# Autodesk Inventor assembly: Direccion
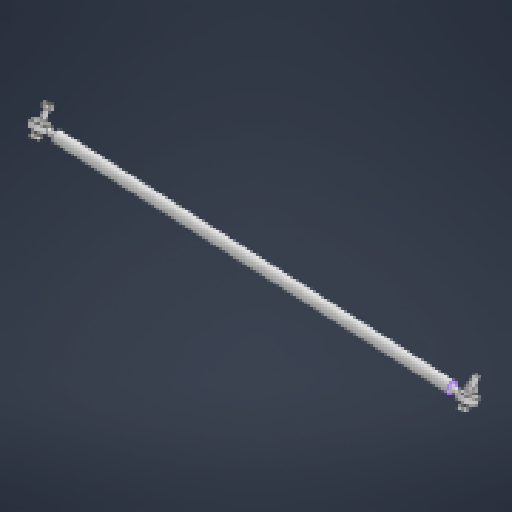
[picture p0: Inventor's stored thumbnail of the model, 512x512]
Saved by Autodesk Inventor 2024 (Build 280153000, 153)
## iProperties
Created: 2023-01-20
Part Number: Direccion
Document SubType Name: Assembly
Designer: juanj
Sending System: Autodesk Inventor 2023
Preprocessor: ST-DEVELOPER v19
Title: C:\Users\juanj\OneDrive\Documentos\Unisabana\Shell\C23 DESING\Dirección\Direccion.stp
Author: juanj
## Documents named in this file (5)
- C:\Users\juanj\Documents\Documentos\Unisabana\Shell\A23[F]\PFA23[F]\D23[F].iam
- C:\Users\juanj\Documents\Documentos\Unisabana\Shell\A23[F]\PWC\BarraAckerman.ipt
- C:\Users\juanj\Documents\Documentos\Unisabana\Shell\A23[F]\PWC\Rotula.ipt
- C:\Users\juanj\Documents\Documentos\Unisabana\Shell\A23[F]\PWC\Tornillo.ipt
- C:\Users\juanj\Documents\Documentos\Unisabana\Shell\A23[F]\PWC\Tuerca.ipt
## Components (7 placed, 4 different names)
1. BarraAckerman:1 — Insert:1, Insert:4
2. Rotula:1 — Insert:1, Insert:2, Insert:3
3. Tornillo:1 — Insert:5, Angle:1
4. Tornillo:2 — Insert:2, Angle:1
5. Tuerca:1 — Insert:6
6. Tuerca:2 — Insert:3
7. Rotula:2 — Insert:4, Insert:5, Insert:6
## Relationships (7: Insert 6, Angle 1)
- Insert:1 (-15 mm): BarraAckerman:1 ↔ Rotula:1
- Insert:2: Rotula:1 ↔ Tornillo:2
- Insert:3 (10 mm): Rotula:1 ↔ Tuerca:2
- Insert:4 (-15 mm): BarraAckerman:1 ↔ Rotula:2
- Insert:5: Tornillo:1 ↔ Rotula:2
- Insert:6 (10 mm): Tuerca:1 ↔ Rotula:2
- Angle:1 (0 deg): Tornillo:1 ↔ Tornillo:2
